# Autodesk Inventor assembly: BuchsenLeiste12
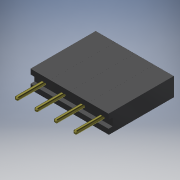
[picture p0: Inventor's stored thumbnail of the model, 180x180]
Saved by Autodesk Inventor 2017.3 (Build 213257000, 257)
## iProperties
Part Number: BuchsenLeiste12
Material: Generisch
Document SubType Name: Assembly
Designer: Enno
Author: Enno
## Documents named in this file (2)
- C:\Users\Enno\Desktop\IMU_Motion_Classification\Adafruit_Feather\CAD\stiftleiste_male-1.snapshot.20\Weib\Gerade\BuchsenLeiste12.iam
- C:\Users\Enno\Desktop\IMU_Motion_Classification\Adafruit_Feather\CAD\stiftleiste_male-1.snapshot.20\Weib\Gerade\Buchsenleiste_female.ipt
## Components (12 placed, 1 different names)
1. Buchsenleiste_female:1 — Passend:1, Passend:2, Passend:3
2. Buchsenleiste_female:2 — Passend:1, Passend:2, Passend:3, Passend:4, Passend:5, Passend:6
3. Buchsenleiste_female:3 — Passend:4, Passend:5, Passend:6, Passend:7, Passend:8, Passend:9
4. Buchsenleiste_female:4 — Passend:7, Passend:8, Passend:9, Passend:10, Passend:11, Passend:12
5. Buchsenleiste_female:5 — Passend:10, Passend:11, Passend:12, Passend:13, Passend:14, Passend:15
6. Buchsenleiste_female:6 — Passend:13, Passend:14, Passend:15, Passend:16, Passend:17, Passend:18
7. Buchsenleiste_female:7 — Passend:16, Passend:17, Passend:18, Passend:19, Passend:20, Passend:21
8. Buchsenleiste_female:8 — Passend:19, Passend:20, Passend:21, Passend:22, Passend:23, Passend:24
9. Buchsenleiste_female:9 — Passend:22, Passend:23, Passend:24, Passend:25, Passend:26, Passend:27
10. Buchsenleiste_female:10 — Passend:25, Passend:26, Passend:27, Passend:28, Passend:29, Passend:30
11. Buchsenleiste_female:11 — Passend:28, Passend:29, Passend:30, Passend:31, Passend:32, Passend:33
12. Buchsenleiste_female:12 — Passend:31, Passend:32, Passend:33
## Relationships (33: Mate 33)
- Passend:1 [Mate]: Buchsenleiste_female:1 ↔ Buchsenleiste_female:2
- Passend:2 [Mate]: Buchsenleiste_female:1 ↔ Buchsenleiste_female:2
- Passend:3 [Mate]: Buchsenleiste_female:1 ↔ Buchsenleiste_female:2
- Passend:4 [Mate]: Buchsenleiste_female:2 ↔ Buchsenleiste_female:3
- Passend:5 [Mate]: Buchsenleiste_female:2 ↔ Buchsenleiste_female:3
- Passend:6 [Mate]: Buchsenleiste_female:2 ↔ Buchsenleiste_female:3
- Passend:7 [Mate]: Buchsenleiste_female:3 ↔ Buchsenleiste_female:4
- Passend:8 [Mate]: Buchsenleiste_female:3 ↔ Buchsenleiste_female:4
- Passend:9 [Mate]: Buchsenleiste_female:3 ↔ Buchsenleiste_female:4
- Passend:10 [Mate]: Buchsenleiste_female:4 ↔ Buchsenleiste_female:5
- Passend:11 [Mate]: Buchsenleiste_female:4 ↔ Buchsenleiste_female:5
- Passend:12 [Mate]: Buchsenleiste_female:4 ↔ Buchsenleiste_female:5
- Passend:13 [Mate]: Buchsenleiste_female:5 ↔ Buchsenleiste_female:6
- Passend:14 [Mate]: Buchsenleiste_female:5 ↔ Buchsenleiste_female:6
- Passend:15 [Mate]: Buchsenleiste_female:5 ↔ Buchsenleiste_female:6
- Passend:16 [Mate]: Buchsenleiste_female:6 ↔ Buchsenleiste_female:7
- Passend:17 [Mate]: Buchsenleiste_female:6 ↔ Buchsenleiste_female:7
- Passend:18 [Mate]: Buchsenleiste_female:6 ↔ Buchsenleiste_female:7
- Passend:19 [Mate]: Buchsenleiste_female:7 ↔ Buchsenleiste_female:8
- Passend:20 [Mate]: Buchsenleiste_female:7 ↔ Buchsenleiste_female:8
- Passend:21 [Mate]: Buchsenleiste_female:7 ↔ Buchsenleiste_female:8
- Passend:22 [Mate]: Buchsenleiste_female:8 ↔ Buchsenleiste_female:9
- Passend:23 [Mate]: Buchsenleiste_female:8 ↔ Buchsenleiste_female:9
- Passend:24 [Mate]: Buchsenleiste_female:8 ↔ Buchsenleiste_female:9
- Passend:25 [Mate]: Buchsenleiste_female:9 ↔ Buchsenleiste_female:10
- Passend:26 [Mate]: Buchsenleiste_female:9 ↔ Buchsenleiste_female:10
- Passend:27 [Mate]: Buchsenleiste_female:9 ↔ Buchsenleiste_female:10
- Passend:28 [Mate]: Buchsenleiste_female:10 ↔ Buchsenleiste_female:11
- Passend:29 [Mate]: Buchsenleiste_female:10 ↔ Buchsenleiste_female:11
- Passend:30 [Mate]: Buchsenleiste_female:10 ↔ Buchsenleiste_female:11
- Passend:31 [Mate]: Buchsenleiste_female:11 ↔ Buchsenleiste_female:12
- Passend:32 [Mate]: Buchsenleiste_female:11 ↔ Buchsenleiste_female:12
- Passend:33 [Mate]: Buchsenleiste_female:11 ↔ Buchsenleiste_female:12
